# Autodesk Inventor assembly: s-assy-motor-wrist3
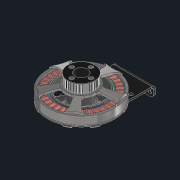
[picture p0: Inventor's stored thumbnail of the model, 180x180]
Saved by Autodesk Inventor 2022 (Build 260153000, 153)
## iProperties
Created: 2021-07-15
Part Number: s-assy-motor-wrist3
Document SubType Name: Assembly
Designer: yuta0
Author: yuta0
## Documents named in this file (9)
- C:\Users\yuta0\Documents\GitHub\catchrobo_hardware\assy-robot\s-assy-motor-wrist3.iam
- C:\Users\yuta0\Documents\GitHub\catchrobo_hardware\assy-robot\base12.ipt
- C:\Users\yuta0\Documents\GitHub\catchrobo_hardware\assy-robot\ex8108.iam
- C:\Users\yuta0\Documents\GitHub\catchrobo_hardware\assy-robot\CBSTNR3-16.ipt
- C:\Users\yuta0\Documents\GitHub\catchrobo_hardware\assy-robot\s-assy-unit-magnet.iam
- C:\Users\yuta0\Documents\GitHub\catchrobo_hardware\assy-robot\steel_plate5.ipt
- C:\Users\yuta0\Documents\GitHub\catchrobo_hardware\assy-robot\s-assy-unit-encoder.iam
- C:\Users\yuta0\Documents\GitHub\catchrobo_hardware\assy-robot\CB4-6.ipt
- C:\Users\yuta0\Documents\GitHub\catchrobo_hardware\assy-robot\s-assy-driver.iam
## Components (14 placed, 8 different names)
1. ex8108:1 [sub-assembly] — メイト:1, メイト:9, メイト:10, メイト:11, メイト:27, メイト:29, メイト:32, メイト:33, メイト:34, メイト:39
2. s-assy-unit-magnet:1 [sub-assembly] — メイト:9, メイト:10, メイト:11
3. steel_plate5:1 — メイト:27, メイト:28, メイト:29, メイト:30, メイト:31, メイト:37, メイト:38, メイト:40, メイト:41
4. s-assy-unit-encoder:1 [sub-assembly] — メイト:26, メイト:30, メイト:31
5. base12:1 — メイト:32, メイト:33, メイト:34, メイト:35, メイト:36
6. s-assy-driver:1 [sub-assembly] — メイト:39, メイト:40, メイト:41
7. CBSTNR3-16:1 — メイト:35, メイト:36
8. CB4-6:1 — メイト:37, メイト:38
9. CBSTNR3-16:2
10. CB4-6:2
11. CBSTNR3-16:3
12. CB4-6:3
13. CBSTNR3-16:4
14. CB4-6:4
## Component patterns: (4 elements, first: CBSTNR3-16:1 + CB4-6:1)
## Relationships (20: Mate 20)
- メイト:1 [Mate]: ex8108:1
- メイト:9 [Mate]: ex8108:1 ↔ s-assy-unit-magnet:1
- メイト:10 [Mate]: ex8108:1 ↔ s-assy-unit-magnet:1
- メイト:11 [Mate]: ex8108:1 ↔ s-assy-unit-magnet:1
- メイト:26 [Mate]: s-assy-unit-encoder:1
- メイト:27 [Mate]: ex8108:1 ↔ steel_plate5:1
- メイト:28 [Mate]: steel_plate5:1
- メイト:29 [Mate]: ex8108:1 ↔ steel_plate5:1
- メイト:30 [Mate]: steel_plate5:1 ↔ s-assy-unit-encoder:1
- メイト:31 [Mate]: steel_plate5:1 ↔ s-assy-unit-encoder:1
- メイト:32 [Mate]: ex8108:1 ↔ base12:1
- メイト:33 [Mate]: ex8108:1 ↔ base12:1
- メイト:34 [Mate]: ex8108:1 ↔ base12:1
- メイト:35 [Mate]: base12:1 ↔ CBSTNR3-16:1
- メイト:36 [Mate]: base12:1 ↔ CBSTNR3-16:1
- メイト:37 [Mate]: steel_plate5:1 ↔ CB4-6:1
- メイト:38 [Mate]: steel_plate5:1 ↔ CB4-6:1
- メイト:39 [Mate]: ex8108:1 ↔ s-assy-driver:1
- メイト:40 [Mate]: steel_plate5:1 ↔ s-assy-driver:1
- メイト:41 [Mate]: steel_plate5:1 ↔ s-assy-driver:1
